# Autodesk Inventor assembly: Wheel on a Stick
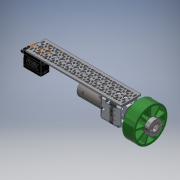
[picture p0: Inventor's stored thumbnail of the model, 180x180]
Saved by Autodesk Inventor 2018 (Build 220112000, 112)
## iProperties
Created: 2020-01-28
Part Number: Wheel on a Stick
Document SubType Name: Assembly
Designer: maste
Author: maste
## Documents named in this file (7)
- C:\Users\maste\OneDrive\Documents\GitHub\2020CAD\Control panel spinny boi\Main Assembly File\Wheel on a Stick.iam
- C:\Users\maste\OneDrive\Documents\GitHub\2020CAD\Control panel spinny boi\Part Files\am-3945 3IN 500Hex Compliant Wheel VER 3.ipt
- C:\Users\maste\OneDrive\Documents\GitHub\2020CAD\Control panel spinny boi\Part Files\am-1526 500Hex HD Collar Clamp.iam
- C:\Users\maste\OneDrive\Documents\GitHub\2020CAD\Control panel spinny boi\Part Files\REV-41-1097.iam
- C:\Users\maste\OneDrive\Documents\GitHub\2020CAD\Control panel spinny boi\Part Files\VersaPlanetary_Lite_0_Stage_3_8_Hex.iam
- C:\Users\maste\OneDrive\Documents\GitHub\2020CAD\Control panel spinny boi\Part Files\REV-41-1787.ipt
- C:\Users\maste\OneDrive\Documents\GitHub\2020CAD\Control panel spinny boi\Part Files\Clamping_Shaft_Collar_-_3_8_Hex_ID_217-2739.ipt
## Components (6 placed, 6 different names)
1. am-3945 3IN 500Hex Compliant Wheel VER 3:1 — Mate:5, Mate:10, Mate:11, Mate:12
2. am-1526 500Hex HD Collar Clamp:1 [sub-assembly] — Mate:5, Mate:12
3. REV-41-1097:1 [sub-assembly] — Mate:6, Mate:7, Mate:8
4. VersaPlanetary_Lite_0_Stage_3_8_Hex:1 [sub-assembly] — Flush:1, Mate:9, Flush:2, Mate:10, Mate:11
5. REV-41-1787:1 — Mate:6, Mate:7, Mate:8, Flush:1, Mate:9, Flush:2
6. Clamping_Shaft_Collar_-_3_8_Hex_ID_217-2739:1
## Relationships (10: Mate 8, Flush 2)
- Mate:5: am-3945 3IN 500Hex Compliant Wheel VER 3:1 ↔ am-1526 500Hex HD Collar Clamp:1
- Mate:6: REV-41-1097:1 ↔ REV-41-1787:1
- Mate:7: REV-41-1097:1 ↔ REV-41-1787:1
- Mate:8: REV-41-1097:1 ↔ REV-41-1787:1
- Flush:1: VersaPlanetary_Lite_0_Stage_3_8_Hex:1 ↔ REV-41-1787:1
- Mate:9: VersaPlanetary_Lite_0_Stage_3_8_Hex:1 ↔ REV-41-1787:1
- Flush:2: VersaPlanetary_Lite_0_Stage_3_8_Hex:1 ↔ REV-41-1787:1
- Mate:10: am-3945 3IN 500Hex Compliant Wheel VER 3:1 ↔ VersaPlanetary_Lite_0_Stage_3_8_Hex:1
- Mate:11: am-3945 3IN 500Hex Compliant Wheel VER 3:1 ↔ VersaPlanetary_Lite_0_Stage_3_8_Hex:1
- Mate:12: am-3945 3IN 500Hex Compliant Wheel VER 3:1 ↔ am-1526 500Hex HD Collar Clamp:1
